# Autodesk Inventor assembly: 6in traction wheel assy
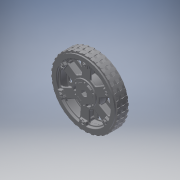
[picture p0: Inventor's stored thumbnail of the model, 180x180]
Saved by Autodesk Inventor 2016 (Build 200138000, 138)
## iProperties
Created: 2013-12-10
Part Number: 6in traction wheel assy
Description: STEP AP214
Document SubType Name: Assembly
Designer: blake
Sending System: SolidWorks 2013
Preprocessor: SwSTEP 2.0
Title: 217-2860-STEP.STEP
Revision Number: ANY
## Documents named in this file (4)
- C:\Users\blake\Documents\24 hour CAD\engineering library\hardware\wheels\6in traction wheel assy.iam
- C:\Users\blake\Documents\24 hour CAD\engineering library\hardware\wheels\6in tire\217-2860-001 Rev3.ipt
- C:\Users\blake\Documents\24 hour CAD\engineering library\hardware\wheels\6in tire\6in traction wheel.iam
- C:\Users\blake\Documents\24 hour CAD\engineering library\hardware\wheels\217-2592-STEP-20140805.ipt
## Components (4 placed, 4 different names)
1. 217-2860-001 Rev3_1 — Mate:2, Mate:4, Mate:10
2. 6in traction wheel:1 [sub-assembly] — Mate:2, Mate:3, Mate:4, Mate:5, Mate:6, Mate:7, Mate:8, Mate:9, Mate:10
3. 217-2860-001 Rev3:2 — Mate:3, Mate:5, Mate:9
4. 217-2592-STEP-20140805:1 — Mate:6, Mate:7, Mate:8
## Relationships (9: Mate 9)
- Mate:2: 217-2860-001 Rev3_1 ↔ 6in traction wheel:1
- Mate:3: 6in traction wheel:1 ↔ 217-2860-001 Rev3:2
- Mate:4: 217-2860-001 Rev3_1 ↔ 6in traction wheel:1
- Mate:5: 6in traction wheel:1 ↔ 217-2860-001 Rev3:2
- Mate:6: 6in traction wheel:1 ↔ 217-2592-STEP-20140805:1
- Mate:7: 6in traction wheel:1 ↔ 217-2592-STEP-20140805:1
- Mate:8: 6in traction wheel:1 ↔ 217-2592-STEP-20140805:1
- Mate:9: 6in traction wheel:1 ↔ 217-2860-001 Rev3:2
- Mate:10: 217-2860-001 Rev3_1 ↔ 6in traction wheel:1
